# Autodesk Inventor assembly: nozzle-assembly_MIR
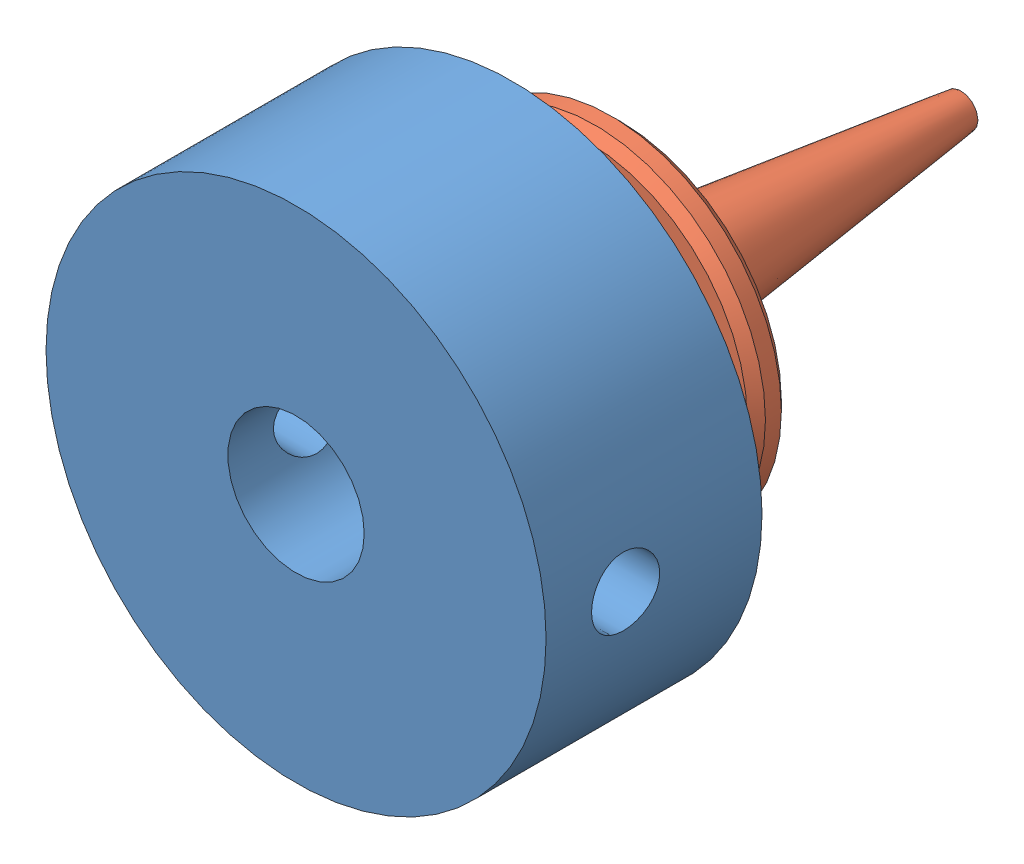
[picture p0: shaded view drawn from the part files that the assembly names]
Saved by Autodesk Inventor 2016 (Build 200138000, 138)
## iProperties
Created: 2015-05-09
Part Number: nozzle-assembly_MIR
Document SubType Name: Assembly
Designer: as
Mass: 27.77 g
Surface Area: 31.6175 cm^2
Volume: 3.41623 cm^3
Density: 8.12884 g/cm^3
Author: ax
## Documents named in this file (3)
- C:\Users\as\Documents\Inventor\mintplacer-export\nozzle-assembly_MIR.iam
- C:\Users\as\Documents\Inventor\mintplacer-export\nozzle-base_MIR.ipt
- C:\Users\as\Documents\Inventor\mintplacer-export\nozzle-tip1-0402_MIR.ipt
## Components (2 placed, 2 different names)
1. nozzle-base_MIR:1 — Flush:1
2. nozzle-tip1-0402_MIR:1 — Flush:1
## Relationships (1: Mate 1)
- Flush:1 [Mate]: nozzle-base_MIR:1 ↔ nozzle-tip1-0402_MIR:1
